# Autodesk Inventor assembly: ASY GBK 3210 central wall shield 4
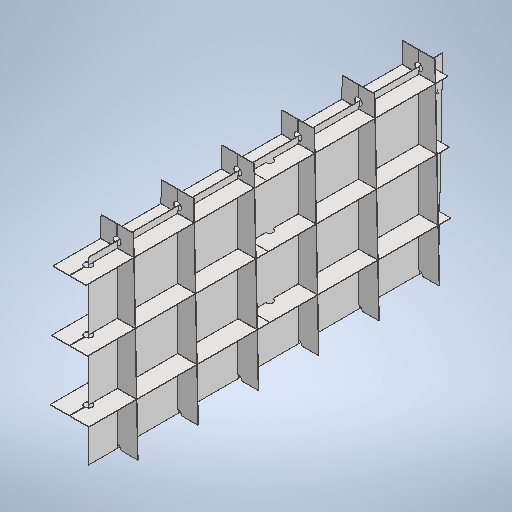
[picture p0: Inventor's stored thumbnail of the model, 512x512]
Saved by Autodesk Inventor 2026 (Build 300175000, 175)
## iProperties
Created: 2026-05-19
Part Number: ASY GBK 3210 central wall shield 4
Document SubType Name: Assembly
Designer: pokla
Mass: 152628 g
Surface Area: 99280.6 cm^2
Volume: 19443.1 cm^3
Density: 7.85 g/cm^3
Author: admin
## Documents named in this file (7)
- C:\Users\pokla\Documents\Inventor\GBK-Gubkinskiy\ASY GBK 3210 central wall shield 4.iam
- C:\Users\pokla\Documents\Inventor\GBK-Gubkinskiy\GBK 3214 stringer 4.ipt
- C:\Users\pokla\Documents\Inventor\GBK-Gubkinskiy\GBK 3215 stringer 5.ipt
- C:\Users\pokla\Documents\Inventor\GBK-Gubkinskiy\GBK 3216 stringer 6.ipt
- C:\Users\pokla\Documents\Inventor\GBK-Gubkinskiy\GBK 3214 shield 4.ipt
- C:\Users\pokla\Documents\Inventor\GBK-Gubkinskiy\GBK 3212 central second rib.ipt
- C:\Users\pokla\Documents\Inventor\GBK-Gubkinskiy\GBK 0101 main rib.ipt
## Components (25 placed, 6 different names)
1. GBK 3214 stringer 4.ipt:1 — Жесткий:1, Жесткий:10
2. GBK 3215 stringer 5.ipt:1 — Жесткий:2, Жесткий:11
3. GBK 3216 stringer 6.ipt:1 — Жесткий:3, Жесткий:12
4. GBK 3214 stringer 4.ipt:2 — Жесткий:6, Жесткий:7
5. GBK 3215 stringer 5.ipt:2 — Жесткий:5, Жесткий:8
6. GBK 3216 stringer 6.ipt:2 — Жесткий:4, Жесткий:9
7. GBK 3214 shield 4.ipt:1 — Совмещение:8, Совмещение:7, Заподлицо:6, Совмещение:5, Заподлицо:7, Совмещение:6, Заподлицо:8
8. GBK 3214 stringer 4.ipt:3 — Жесткий:7
9. GBK 3215 stringer 5.ipt:3 — Жесткий:8
10. GBK 3216 stringer 6.ipt:3 — Жесткий:9, Заподлицо:8
11. GBK 3214 stringer 4.ipt:4 — Жесткий:10
12. GBK 3215 stringer 5.ipt:4 — Жесткий:11
13. GBK 3216 stringer 6.ipt:4 — Жесткий:12
14. GBK 3212 central second rib.ipt:1 — Совмещение:5, Заподлицо:4, Жесткий:6, Жесткий:5, Жесткий:4, Совмещение:5, Заподлицо:7
15. GBK 3212 central second rib.ipt:2 — Совмещение:6, Заподлицо:4, Жесткий:1, Жесткий:2, Жесткий:3, Совмещение:6
16. GBK 3212 central second rib:3
17. GBK 3212 central second rib:4
18. GBK 3212 central second rib:5
19. GBK 3212 central second rib:6
20. GBK 3212 central second rib:7
21. GBK 3212 central second rib:8
22. GBK 3212 central second rib:9
23. GBK 3212 central second rib:10
24. GBK 3212 central second rib:11
25. GBK 3212 central second rib:12
## Component patterns: (6 elements, first: GBK 3212 central second rib.ipt:1 + GBK 3212 central second rib.ipt:2)
## Relationships (22: WeldJoint 12, Mate 6, Flush 4)
- Совмещение:6 [Mate]: GBK 3212 central second rib.ipt:2
- Совмещение:5 [Mate]: GBK 3212 central second rib.ipt:1
- Заподлицо:4 [Flush]: GBK 3212 central second rib.ipt:1 ↔ GBK 3212 central second rib.ipt:2
- Совмещение:8 [Mate]: GBK 3214 shield 4.ipt:1
- Совмещение:7 [Mate]: GBK 3214 shield 4.ipt:1
- Жесткий:1 [WeldJoint] (4 mm): GBK 3214 stringer 4.ipt:1 ↔ GBK 3212 central second rib.ipt:2
- Жесткий:2 [WeldJoint] (4 mm): GBK 3215 stringer 5.ipt:1 ↔ GBK 3212 central second rib.ipt:2
- Жесткий:3 [WeldJoint] (4 mm): GBK 3216 stringer 6.ipt:1 ↔ GBK 3212 central second rib.ipt:2
- Жесткий:6 [WeldJoint] (4 mm): GBK 3214 stringer 4.ipt:2 ↔ GBK 3212 central second rib.ipt:1
- Жесткий:5 [WeldJoint] (4 mm): GBK 3215 stringer 5.ipt:2 ↔ GBK 3212 central second rib.ipt:1
- Жесткий:4 [WeldJoint] (4 mm): GBK 3216 stringer 6.ipt:2 ↔ GBK 3212 central second rib.ipt:1
- Заподлицо:6 [Flush]: GBK 3214 shield 4.ipt:1
- Совмещение:5 [Mate]: GBK 3214 shield 4.ipt:1 ↔ GBK 3212 central second rib.ipt:1
- Заподлицо:7 [Flush]: GBK 3214 shield 4.ipt:1 ↔ GBK 3212 central second rib.ipt:1
- Жесткий:7 [WeldJoint] (1 mm): GBK 3214 stringer 4.ipt:2 ↔ GBK 3214 stringer 4.ipt:3
- Жесткий:8 [WeldJoint] (1 mm): GBK 3215 stringer 5.ipt:2 ↔ GBK 3215 stringer 5.ipt:3
- Жесткий:9 [WeldJoint] (1 mm): GBK 3216 stringer 6.ipt:2 ↔ GBK 3216 stringer 6.ipt:3
- Жесткий:10 [WeldJoint] (1 mm): GBK 3214 stringer 4.ipt:1 ↔ GBK 3214 stringer 4.ipt:4
- Жесткий:11 [WeldJoint] (1 mm): GBK 3215 stringer 5.ipt:1 ↔ GBK 3215 stringer 5.ipt:4
- Жесткий:12 [WeldJoint] (1 mm): GBK 3216 stringer 6.ipt:1 ↔ GBK 3216 stringer 6.ipt:4
- Совмещение:6 [Mate]: GBK 3214 shield 4.ipt:1 ↔ GBK 3212 central second rib.ipt:2
- Заподлицо:8 [Flush] (155 mm): GBK 3214 shield 4.ipt:1 ↔ GBK 3216 stringer 6.ipt:3
## Named parameters: Шаг_шпангоутов = 496.66667 mm
